# Autodesk Inventor assembly: still pipe
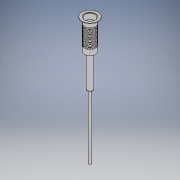
[picture p0: Inventor's stored thumbnail of the model, 180x180]
Saved by Autodesk Inventor 2018 (Build 220112000, 112)
## iProperties
Created: 2019-01-14
Part Number: still pipe
Document SubType Name: Assembly
Designer: Admin
Author: Admin
## Documents named in this file (4)
- C:\Users\Admin\Documents\Cryostat\CAD\still pipe.iam
- C:\Users\Admin\Documents\Cryostat\CAD\KF50 bellows.ipt
- C:\Users\Admin\Documents\Cryostat\CAD\still pipe small.iam.ipt
- still pipe small.iam
## Components (2 placed, 2 different names)
1. KF50 bellows:1 — Mate:1
2. still pipe small.iam:1 — Mate:1
## Relationships (1: Mate 1)
- Mate:1: KF50 bellows:1 ↔ still pipe small.iam:1
